# Autodesk Inventor assembly: Screen_Case
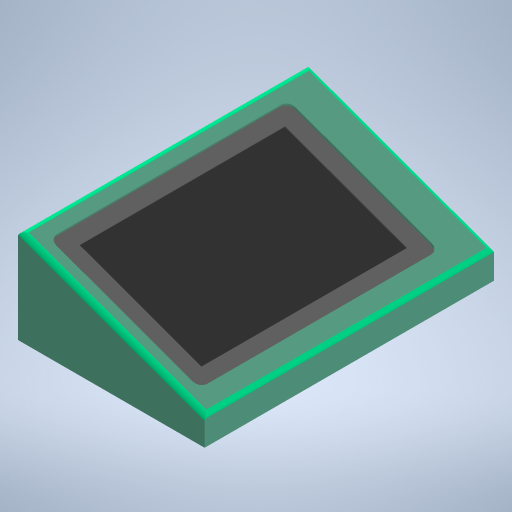
[picture p0: Inventor's stored thumbnail of the model, 512x512]
Saved by Autodesk Inventor 2024 (Build 280153000, 153)
## iProperties
Created: 2024-02-15
Part Number: Screen_Case
Document SubType Name: Assembly
Designer: fabiancastano
Author: fabiancastano
## Documents named in this file (3)
- C:\GitHub\PulseLaserPrj\CaseDesign\Case_parts\Screen_Case.iam
- C:\GitHub\PulseLaserPrj\CaseDesign\BaseFiles\LCD_10.1\LCD_10.1.iam
- C:\GitHub\PulseLaserPrj\CaseDesign\Case_parts\Screen_Support.ipt
## Components (2 placed, 2 different names)
1. LCD_10.1:1 [sub-assembly] — Mate:1, Mate:2, Mate:3
2. Screen_Support:1 — Mate:1, Mate:2, Mate:3
## Relationships (3: Mate 3)
- Mate:1: LCD_10.1:1 ↔ Screen_Support:1
- Mate:2: LCD_10.1:1 ↔ Screen_Support:1
- Mate:3: LCD_10.1:1 ↔ Screen_Support:1
